# Autodesk Inventor assembly: 041.5-DXP
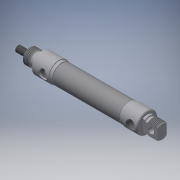
[picture p0: Inventor's stored thumbnail of the model, 180x180]
Saved by Autodesk Inventor 2019 (Build 230136000, 136)
## iProperties
Category: PARTsolutions
Company: BIMBA
Created: 2019-01-29
Part Number: 041.5-DXP
Catalog Web Link: www.cadenas.de
Description: Original Line Standard Air Cylinders-Standard Air Cylinders
Vendor: BIMBA
Document SubType Name: Assembly
Designer: psadmin
Manufacturer: BIMBA
Mass: 39.857 g
Surface Area: 247.284 cm^2
Volume: 39.857 cm^3
Density: 1 g/cm^3
PSOL_IDENT_0: {$CADENAS_DATA\23d-libs\bimba\bimba\bimba_imperial\bimba_full_line\original_line_cylinders\standard_
PSOL_IDENT_1: air_cylinders\standard_air_cylinder_asmtab.prj},326 {VTYP=3D},{STYP=ASSTAB},{NB=041.5-DXP},{LINA=041
PSOL_IDENT_2: .5-DXP},{NN=Original Line Standard Air Cylinders},{DATE=21.03.2018 14:31:21},{GEOMDATE=19.03.2018 11
PSOL_IDENT_3: :39:15},{VERSION=},{LINEID=50},{WBVAR=STROKE,ACTING,MNT,DER,NR,BM,CO,OO,VO,M,EE,EEL,K,Q,Y,G,T,HL,B,H
PSOL_IDENT_4: ,SER,SR,NT,W,STPT1,STPT2,STPT3,STPT4,MB,PB,PRC,TB,MN},{WBNUMERIC=STROKE,EEL}  {NB=041.5-DXP},{LINA=0
PSOL_IDENT_5: 41.5-DXP},{KT=DUMMY},{PN=041.5-DXP},{PNC=041.5-DXP},{PNA=(NO ACCESSORIES)},{DASH=-},{BORE1=0.7500000
PSOL_IDENT_6: 0},{BORE=3/4\" (04)},{BOREPN=04},{STROKE=1.500},{STROKEALG=[0.011:50/0.001]},{STROKE1=1.500},{ACTING=
PSOL_IDENT_7: D},{ACTINGALG= '' , 'Single Acting (SA)' , 'R' , 'Reverse Single Acting (SA)' , 'D' , 'Double Acting
PSOL_IDENT_8: (SA)' },{ACTINGPN=D},{MNT=XP},{MNTALG= '' , 'Front Nose Mounting (SA)' , 'P' , 'Rear Pivot Mounting
PSOL_IDENT_9: (SA)' , 'XP' , 'Double End or Pivot Mounting (SA)' , 'X' , 'Double End Mounting (SA)' , 'BF' , 'Fro
PSOL_IDENT_10: nt Block Mounting (SA)' , 'BR' , 'Rear Block Mounting for Vertical Positioning (SA)' , 'BFT' , 'Fron
PSOL_IDENT_11: t Block Trunnion Mounting (SA)' , 'BRT' , 'Rear Block Trunnion Mounting (SA)' },{TYPE=},{MNTPN=XP},{
PSOL_IDENT_12: DER=},{DERALG= '' , 'N/A' },{NR=},{NRALG= '' , 'N/A' },{NRPN=},{BM=},{BMALG= '' , 'N/A' },{BMPN=},{C
PSOL_IDENT_13: O=},{COALG= '' , 'N/A' },{OO=},{OOALG= '', 'N/A' },{OOPN=},{VO=Z},{VOALG= 'Z' , 'N/A' },{VOPN=},{OOV
PSOL_IDENT_14: OPN=},{M=},{MALG= '', 'Without Magnet', 'M', 'With Magnet' },{EE=},{EEL=0.000},{EEMAX=48.5000},{EEAL
PSOL_IDENT_15: G= '', 'Without Extra Extension', 'EE', 'With Extra Extension' },{EELALG=0},{EEPN=},{EEPN1=0.000},{K=
PSOL_IDENT_16: },{KALG= '', 'Standard' , 'K' , 'Ports Rotated 90deg K' },{KPN=},{Q=},{QALG= '' , 'N/A' },{QPN=},{Y=
PSOL_IDENT_17: },{YALG= '' , 'Without Pivot Bushing' , 'Y' , 'With Pivot Bushing' },{YPN=},{YCON=},{F=},{FALG= '', '
PSOL_IDENT_18: Non-Coated (Standard)', 'F', 'Molycoated' },{FPN=},{G=},{GPN=},{GPN99=},{T=},{TALG= '' , 'Standard -
PSOL_IDENT_19: 20° to 200°F (-29° to 95°C)' , 'N' , 'Low Temperature' , 'V' , 'High Temperature' },{NPN=},{VPN=},{H
PSOL_IDENT_20: L=},{HLALG= '' , 'Without Low Pressure Hydraulic' , 'HL' , 'With Low Pressure Hydraulic' },{B=},{BAL
PSOL_IDENT_21: G= '', 'W/out Bumpers' , 'B' , 'W/ Bumpers' },{BPN=},{H=},{HALG= '', 'N/A' },{HPN=},{SER=},{SERALG= ''
PSOL_IDENT_22: , 'Without Spring Extend/Return' , 'JS' , 'With Spring Return' , 'JR' , 'With Spring Extend' },{SR=
PSOL_IDENT_23: },{SRALG= '' , 'Standard Stainless Steel' },{SRPN=},{SRCON=0},{NT=},{NTPN=},{W=},{WALG= '' , 'Withou
PSOL_IDENT_24: t Wiper' , 'W' , 'With Wiper' },{WPN=},{E=},{EALG= '' , 'Standard Seals/Lube' , 'E' , 'Non-Lube Seal
PSOL_IDENT_25: s/Lube' },{EPN=},{ST=},{STALG= '' , 'N/A' },{STPT1=},{STPT1ALG= '' , 'N/A' },{STPT2=},{STPT2ALG= ''
PSOL_IDENT_26: , 'N/A' },{STPT3=},{STPT3ALG= '' , 'N/A' },{STPT4=},{STPT4ALG= '' , 'N/A' },{STPN=},{MB=},{MBALG= ''
PSOL_IDENT_27: , 'Without Mounting Bracket' , 'F,D-129' , 'D-129 (front)'  , 'R,D-129' , 'D-129 (rear)' , '2x,D-12
PSOL_IDENT_28: 9' , 'D-129 (front & rear)'},{MBPN=},{MBPNALL=D-129},{MBPNALLREAR=D-129},{PB=},{PBALG= '' , 'Without
PSOL_IDENT_29: Pivot Bracket' , 'D-13498-A' , 'D-13498-A' },{PBPN=},{PBPNALL=D-13498-A},{PRC=},{PRCALG= '' , 'W/ou
PSOL_IDENT_30: t Pivot Rod Clevis' , 'F,D-166-3' , 'D-166-3 (front)' },{PRCPN=},{PRCPNALL=D-166-3},{TB=},{TBALG= ''
PSOL_IDENT_31: , 'N/A' },{TBPN=},{TBPNALL=},{MN=},{MNALG= '' , 'N/A' },{MNPN=},{MNCONF=},{MNCONR=},{TLEN=2.7555},{
PSOL_IDENT_32: FRAC=6.2500},{RGCON=},{RGDACCON=R},{RHCON=P},{RHCON1=P},{RHCONON=1},{RHACCON=},{FNUTCON=1},{RNUTCON=
PSOL_IDENT_33: 1},{FNUTPN=D-9},{RNUTPN=D-9},{FNUTTRANS=0.0000},{RNUTTRANS=0.0000},{VHOLECON=0},{A1=1.5940},{A1N=0.8
PSOL_IDENT_34: 750},{A1P=1.5940},{A1B=1.5940},{A4=0.2525},{A4N=0.3130},{A4P=0.2525},{A5=0.0300},{A1H=1.594},{A1NH=0
PSOL_IDENT_35: .5310},{A1PH=1.5940},{A1BH=1.0940},{A1SH=1.2190},{A2H=0.2190},{A2NH=0.2190},{LENGTH=3.7500},{LENGTH1=
PSOL_IDENT_36: 3.7500},{LENGTH2=3.8100},{MUL=1.5000},{MUL11=1.5000},{MUL22=4.035},{MUL33=2.5350},{MUL2=1.5000},{MUL
PSOL_IDENT_37: 211=1.5000},{MUL222=2.6900},{MUL233=1.6900},{SSS=3.0000},{RGLEN=1.3715},{RHLEN=1.1230},{SSS1=2.0000}
PSOL_IDENT_38: ,{A13=1.3120},{DIF=0.0000},{G5=0.6250},{ON=0},{SSADD=0.0000},{BADD=0.0000},{MADD=0.0000},{NVADD=0.00
PSOL_IDENT_39: 00},{TRACKL=2.4655},{TRACKCON=D-74168},{TRIMCON=0},{TRIMCON1=0},{PINCON=D-51},{FSPACE=0.6819},{SPACE=
PSOL_IDENT_40: 0.0589},{TEXT=0.1031},{S1=1.0000},{D1=0.8325},{D1N=0.8050},{D1B=0.8625},{D1P=0.8325},{FA=0.940},{RA=
PSOL_IDENT_41: 0.9400},{PPATH=standard_air_cylinder_asmtpl.prj},{MATALGHTML=<b>Standard Original Line:</b><dl><dt>R
PSOL_IDENT_42: od:</dt><dd>- Stainless Steel</dd><dd>&nbsp;&nbsp;(5/16 9/16 Bores)</dd><dd>- High Strength Carbon S
PSOL_IDENT_43: teel</dd><dd>&nbsp;&nbsp;(3/4 3 Bore)</dd><dd>- Stainless Steel</dd><dd>&nbsp;&nbsp;(X style DXP/DX/
PSOL_IDENT_44: DXDE)</dd><dt>Bearings:</dt><dd>- Sintered Bronze</dd><dt>Body:</dt><dd>- 304 Stainless Steel</dd><d
PSOL_IDENT_45: t>End Caps:</dt><dd>- Aluminum</dd><dt>Seals:</dt><dd>- Buna N</dd></dl>},{ASSCFGPRA=04DXP},{MBPNA=}
PSOL_IDENT_46: ,{MNPNA=},{PRCPNA=},{ASSOPTACC=STPT4},{A=5.25},{HADD=0.0000},{WFL=0.25},{QADD=0.000},{QADD1=0.440},{
PSOL_IDENT_47: TEST=1.0000},{MNTB=},{STDNUTF=1},{STDNUTR=1},{STRK2D=0},{X2D=2},{STROKESW=1.500},{EESW=0.000},{FCD=0
PSOL_IDENT_48: },{BCD=0},{RCD=0},{CUSTADD=0.500},{FT=1/4-28 UNF-2A},{FT1=1/4-28 UNF-2A},{FT2=5/8-18 UNF-2A},{PORT=1
PSOL_IDENT_49: /8 NPT},{FT11=1/2-20 UNF-2A},{FT12=5/8-18 UNF-2A},{B1=}
NN: Original Line Standard Air Cylinders
NT: Standard Male Thread
NB: 041.5-DXP
NBSYN: $PNC.
LINA: 041.5-DXP
PN: 041.5-DXP
PNA: (NO ACCESSORIES)
BORE: 3/4" (04)
STROKE: 1.5
ACTING: Double [D]
MNT: Universal Double End or Rear Pivot [XP]
DER: N/A
NR: N/A
BM: N/A
CO: N/A
OO: N/A
VO: N/A
M: Without Magnet Piston
EE: Standard Rod Extension
EEL: 0
K: Standard
Q: N/A
Y: Standard Pivot Style
G: Standard Grease Lube
T: Standard -20° to 200°F (-29° to 95°C)
HL: Standard 250 PSI Air
B: Without Bumpers
H: N/A
SER: Without Failsafe Spring Extend/Return
SR: Standard Stainless Steel
W: Without Wiper
STPT1: N/A
STPT2: N/A
STPT3: N/A
STPT4: N/A
MB: Without Mounting Bracket
PB: Without Pivot Bracket
PRC: Without Piston Rod Clevis
TB: N/A
MN: N/A
A: 5.25
SUPPLIER: BIMBA
ARTICLENO: 041.5-DXP
BOMINFO: 041.5-DXP
CREATOR: CADENAS GmbH
Title: 041.5-DXP
Author: Cadenas PARTsolutions
Comments: Standard Air Cylinders
## Documents named in this file (6)
- C:\Users\leadere\Documents\GrabCAD\2019 Robot\Imported Components\Pneumatic Cylinders\Cylinders\0.75x1.5 adaptive\0.75x1.5_041_5-DXP.iam
- C:\Users\leadere\Documents\GrabCAD\2019 Robot\Imported Components\Pneumatic Cylinders\Cylinders\0.75x1.5 adaptive\041_5-DXP0000000_0_dummy.ipt
- C:\Users\leadere\Documents\GrabCAD\2019 Robot\Imported Components\Pneumatic Cylinders\Cylinders\0.75x1.5 adaptive\04R000-0_rod_guide.ipt
- C:\Users\leadere\Documents\GrabCAD\2019 Robot\Imported Components\Pneumatic Cylinders\Cylinders\0.75x1.5 adaptive\04R-2_75550.ipt
- C:\Users\leadere\Documents\GrabCAD\2019 Robot\Imported Components\Pneumatic Cylinders\Cylinders\0.75x1.5 adaptive\04P0000_rear_head.ipt
- C:\Users\leadere\Documents\GrabCAD\2019 Robot\Imported Components\Pneumatic Cylinders\Cylinders\0.75x1.5 adaptive\041_5-DXP0000_rod.ipt
## Components (6 placed, 5 different names)
1. 041_5-DXP0000000_0_dummy:1
2. 04R000-0_rod_guide:1
3. 04R-2_75550:1
4. 04P0000_rear_head:1
5. 041_5-DXP0000_rod:1 — Flush:1, Mate:1
6. 041_5-DXP0000_rod:2 — Flush:1, Mate:1
## Relationships (2: Flush 1, Mate 1)
- Flush:1: 041_5-DXP0000_rod:1 ↔ 041_5-DXP0000_rod:2
- Mate:1: 041_5-DXP0000_rod:1 ↔ 041_5-DXP0000_rod:2
